# Autodesk Inventor assembly: DriveTrain
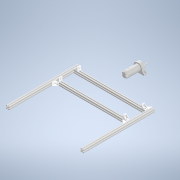
[picture p0: Inventor's stored thumbnail of the model, 180x180]
Saved by Autodesk Inventor 2020.2 (Build 242310000, 310)
## iProperties
Created: 2020-01-29
Part Number: DriveTrain
Document SubType Name: Assembly
Designer: yukin
Author: yukin
## Documents named in this file (5)
- C:\Autodesk\Files\CAD\Robotics 2019-2020\DriveTrain\DriveTrain.iam
- C:\Autodesk\Files\CAD\Robotics 2019-2020\DriveTrain\RevHexMotor\RevHexMotor.iam
- C:\Autodesk\Files\CAD\Robotics 2019-2020\DriveTrain\MotorMount_vCAD.ipt
- C:\Autodesk\Files\CAD\Robotics 2019-2020\DriveTrain\Extrusions\17in.ipt
- C:\Autodesk\Files\CAD\Robotics 2019-2020\DriveTrain\CornerBracket.ipt
## Components (14 placed, 4 different names)
1. RevHexMotor:1 [sub-assembly] — Rotational:1
2. MotorMount_vCAD:1 — Rotational:1
3. 17in:1 — Mate:1, Flush:1, Flush:2, Flush:12, Flush:13, Mate:7, Mate:8, Flush:14, Flush:15, Mate:11, Flush:19, Flush:20
4. 17in:2 — Flush:3, Mate:2, Flush:4, Flush:7, Flush:8, Flush:9, Mate:5, Flush:10, Mate:6, Flush:11, Mate:12
5. CornerBracket:1 — Flush:3, Mate:2, Flush:4, Mate:4
6. CornerBracket:2 — Mate:1, Flush:1, Flush:2, Flush:5, Mate:3, Flush:6
7. 17in:3 — Flush:5, Mate:3, Flush:6, Mate:4, Flush:7
8. CornerBracket:3 — Mate:8, Flush:14, Flush:15
9. CornerBracket:4 — Flush:12, Flush:13, Mate:7
10. CornerBracket:5 — Flush:8, Flush:9, Mate:5
11. CornerBracket:6 — Flush:10, Mate:6, Flush:11
12. 17in:4 — Mate:9, Flush:16, Flush:17, Mate:10, Flush:18, Flush:20
13. CornerBracket:7 — Mate:9, Flush:16, Flush:17, Mate:11, Flush:19
14. CornerBracket:8 — Mate:10, Flush:18, Mate:12
## Relationships (33: Flush 20, Mate 12, RevoluteJoint 1)
- Rotational:1 [RevoluteJoint]: RevHexMotor:1 ↔ MotorMount_vCAD:1
- Mate:1: 17in:1 ↔ CornerBracket:2
- Flush:1: 17in:1 ↔ CornerBracket:2
- Flush:2: 17in:1 ↔ CornerBracket:2
- Flush:3: 17in:2 ↔ CornerBracket:1
- Mate:2: 17in:2 ↔ CornerBracket:1
- Flush:4: 17in:2 ↔ CornerBracket:1
- Flush:5: CornerBracket:2 ↔ 17in:3
- Mate:3: CornerBracket:2 ↔ 17in:3
- Flush:6: CornerBracket:2 ↔ 17in:3
- Mate:4: CornerBracket:1 ↔ 17in:3
- Flush:7: 17in:2 ↔ 17in:3
- Flush:8: 17in:2 ↔ CornerBracket:5
- Flush:9: 17in:2 ↔ CornerBracket:5
- Mate:5: 17in:2 ↔ CornerBracket:5
- Flush:10: 17in:2 ↔ CornerBracket:6
- Mate:6: 17in:2 ↔ CornerBracket:6
- Flush:11: 17in:2 ↔ CornerBracket:6
- Flush:12: 17in:1 ↔ CornerBracket:4
- Flush:13: 17in:1 ↔ CornerBracket:4
- Mate:7: 17in:1 ↔ CornerBracket:4
- Mate:8: 17in:1 ↔ CornerBracket:3
- Flush:14: 17in:1 ↔ CornerBracket:3
- Flush:15: 17in:1 ↔ CornerBracket:3
- Mate:9: 17in:4 ↔ CornerBracket:7
- Flush:16: 17in:4 ↔ CornerBracket:7
- Flush:17: 17in:4 ↔ CornerBracket:7
- Mate:10: 17in:4 ↔ CornerBracket:8
- Flush:18: 17in:4 ↔ CornerBracket:8
- Mate:11: 17in:1 ↔ CornerBracket:7
- Flush:19: 17in:1 ↔ CornerBracket:7
- Mate:12: 17in:2 ↔ CornerBracket:8
- Flush:20: 17in:1 ↔ 17in:4
